# Autodesk Inventor assembly: Pin-connector-angled-4
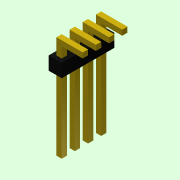
[picture p0: Inventor's stored thumbnail of the model, 180x180]
Saved by Autodesk Inventor 2016 (Build 200138000, 138)
## iProperties
Created: 2015-06-24
Part Number: Pin-connector-angled-4
Document SubType Name: Assembly
Designer: Openlab
Author: Openlab
## Documents named in this file (2)
- D:\Alexey\HS-Spectrophotometer\parts\Common\Pin-connector-angled-4.iam
- D:\Alexey\HS-Spectrophotometer\parts\Common\Pin-connector-angled.ipt
## Components (4 placed, 1 different names)
1. Pin-connector-angled:1 — Mate:1, Flush:1, Flush:6
2. Pin-connector-angled:2 — Mate:1, Mate:2, Flush:1, Flush:2, Flush:5, Flush:6
3. Pin-connector-angled:3 — Mate:2, Mate:3, Flush:2, Flush:3, Flush:4, Flush:5
4. Pin-connector-angled:4 — Mate:3, Flush:3, Flush:4
## Relationships (9: Flush 6, Mate 3)
- Mate:1: Pin-connector-angled:1 ↔ Pin-connector-angled:2
- Mate:2: Pin-connector-angled:2 ↔ Pin-connector-angled:3
- Mate:3: Pin-connector-angled:3 ↔ Pin-connector-angled:4
- Flush:1: Pin-connector-angled:1 ↔ Pin-connector-angled:2
- Flush:2: Pin-connector-angled:2 ↔ Pin-connector-angled:3
- Flush:3: Pin-connector-angled:3 ↔ Pin-connector-angled:4
- Flush:4: Pin-connector-angled:3 ↔ Pin-connector-angled:4
- Flush:5: Pin-connector-angled:2 ↔ Pin-connector-angled:3
- Flush:6: Pin-connector-angled:1 ↔ Pin-connector-angled:2
